# Autodesk Inventor assembly: stand
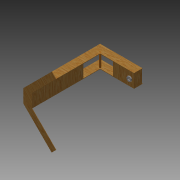
[picture p0: Inventor's stored thumbnail of the model, 180x180]
Saved by Autodesk Inventor 2013 (Build 170138000, 138)
## iProperties
Created: 2014-10-20
Part Number: stand
Document SubType Name: Assembly
Designer: Masta
Author: Masta
## Documents named in this file (10)
- D:\DrOctopus\3D model\stand\stand.iam
- D:\DrOctopus\3D model\stand\stand_plate1.ipt
- D:\DrOctopus\3D model\stand\stand_plate3.ipt
- D:\DrOctopus\3D model\stand\stand_plate4.ipt
- D:\DrOctopus\3D model\stand\base_plate.ipt
- D:\DrOctopus\3D model\stand\Bearing 6006 ZZ - 30x55x13mm.ipt
- D:\DrOctopus\3D model\stand\Thrust Bearing 51106 - 30x47x11mm.ipt
- D:\DrOctopus\3D model\stand\pin.ipt
- D:\DrOctopus\3D model\stand\stand_plate2.ipt
- D:\DrOctopus\3D model\stand\leg.ipt
## Components (10 placed, 9 different names)
1. stand_plate1:1 — Mate:2, Flush:3, Flush:11, Flush:12, Mate:9, Insert:3, Flush:13, Mate:12
2. stand_plate1:2 — Mate:6, Flush:6, Flush:8, Flush:10, Mate:7, Mate:10, Flush:14
3. stand_plate3:1 — Mate:2, Flush:3, Mate:8
4. stand_plate4:2 — Mate:6, Flush:6, Flush:8
5. base_plate:1 — Flush:10, Mate:7, Flush:11, Mate:8, Flush:12, Mate:9, Insert:1, Insert:2
6. Bearing 6006 ZZ - 30x55x13mm:1 — Insert:2
7. Thrust Bearing 51106 - 30x47x11mm:1 — Insert:1
8. pin:1 — Insert:3
9. stand_plate2:1 — Mate:10, Flush:13, Flush:14, Mate:11, Flush:15
10. leg:1 — Mate:11, Flush:15, Mate:12
## Relationships (20: Flush 9, Mate 8, Insert 3)
- Mate:2: stand_plate1:1 ↔ stand_plate3:1
- Flush:3: stand_plate1:1 ↔ stand_plate3:1
- Mate:6: stand_plate1:2 ↔ stand_plate4:2
- Flush:6: stand_plate1:2 ↔ stand_plate4:2
- Flush:8: stand_plate1:2 ↔ stand_plate4:2
- Flush:10: stand_plate1:2 ↔ base_plate:1
- Mate:7: stand_plate1:2 ↔ base_plate:1
- Flush:11: stand_plate1:1 ↔ base_plate:1
- Mate:8: stand_plate3:1 ↔ base_plate:1
- Flush:12: stand_plate1:1 ↔ base_plate:1
- Mate:9: stand_plate1:1 ↔ base_plate:1
- Insert:1: base_plate:1 ↔ Thrust Bearing 51106 - 30x47x11mm:1
- Insert:2: base_plate:1 ↔ Bearing 6006 ZZ - 30x55x13mm:1
- Insert:3: stand_plate1:1 ↔ pin:1
- Mate:10: stand_plate1:2 ↔ stand_plate2:1
- Flush:13: stand_plate1:1 ↔ stand_plate2:1
- Flush:14: stand_plate1:2 ↔ stand_plate2:1
- Mate:11: stand_plate2:1 ↔ leg:1
- Flush:15: stand_plate2:1 ↔ leg:1
- Mate:12: stand_plate1:1 ↔ leg:1
